# Autodesk Inventor assembly: fuse
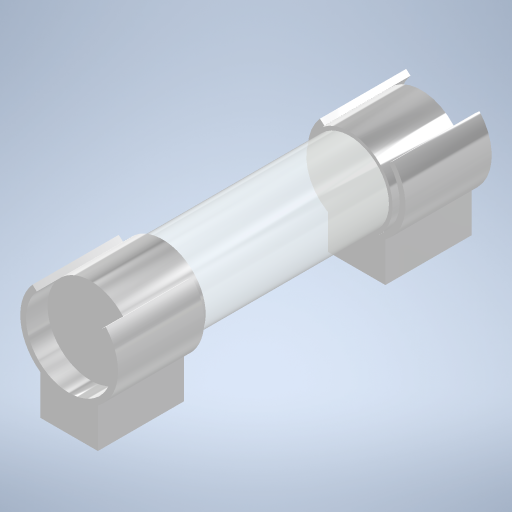
[picture p0: Inventor's stored thumbnail of the model, 512x512]
Saved by Autodesk Inventor 2024.1 (Build 281209000, 209)
## iProperties
Created: 2025-02-19
Part Number: fuse
Document SubType Name: Assembly
Designer: hibik
Author: hibik
## Documents named in this file (3)
- C:\Users\hibik\Documents\Robomech\RESCUE\ORCA\hard\std_parts\fuse.iam
- C:\Users\hibik\Documents\Robomech\RESCUE\ORCA\hard\std_parts\fuse_cover.ipt
- C:\Users\hibik\Documents\Robomech\RESCUE\ORCA\hard\std_parts\fuse_fuse.ipt
## Components (2 placed, 2 different names)
1. fuse_cover:1 — 挿入:1
2. fuse_fuse:1 — 挿入:1
## Relationships (1: Insert 1)
- 挿入:1 [Insert]: fuse_cover:1 ↔ fuse_fuse:1
